# Autodesk Inventor assembly: 部件1
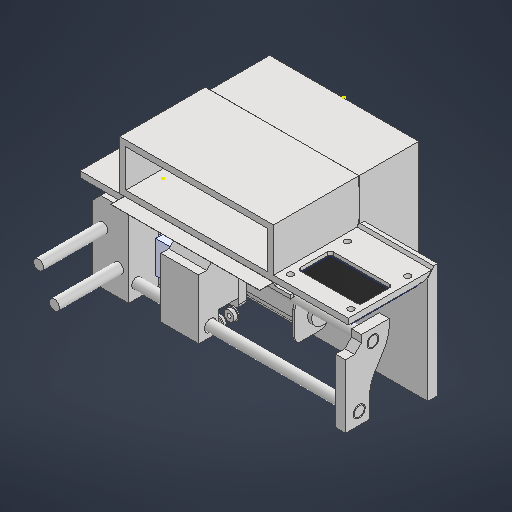
[picture p0: Inventor's stored thumbnail of the model, 512x512]
Saved by Autodesk Inventor 2025 (Build 290162000, 162)
## iProperties
Created: 2025-11-30
Part Number: 部件1
Document SubType Name: Assembly
Designer: XH
Author: XH
## Documents named in this file (11)
- C:\1A_Engineering_files\braille-printer-v2\部件1.iam
- C:\1A_Engineering_files\braille-printer-v2\便签.ipt
- C:\1A_Engineering_files\braille-printer-v2\主体.ipt
- C:\1A_Engineering_files\braille-printer-v2\前舵机位置控制.ipt
- C:\1A_Engineering_files\braille-printer-v2\针头主体.iam
- C:\1A_Engineering_files\braille-printer-v2\钢轴.ipt
- C:\1A_Engineering_files\braille-printer-v2\Y轴杠轴.ipt
- C:\1A_Engineering_files\braille-printer-v2\xy转接连杆.ipt
- C:\1A_Engineering_files\braille-printer-v2\阻挡X轴.ipt
- C:\1A_Engineering_files\braille-printer-v2\AZ-Delivery - OLED13 IIC.ipt
- C:\1A_Engineering_files\braille-printer-v2\大外壳.ipt
## Components (12 placed, 10 different names)
1. 便签:1 — 配合:1, 配合:2
2. 主体:1 — 配合:1, 配合:2, 表面齐平:7, 配合:12, 配合:13, 表面齐平:9, 配合:17, 表面齐平:10, 表面齐平:11
3. 前舵机位置控制:1 — 配合:14, 配合:15, 配合:16, 表面齐平:9
4. 针头主体:1 [sub-assembly] — 配合:4, 配合:5
5. 钢轴:1 — 表面齐平:3, 配合:4, 配合:6, 配合:10
6. 钢轴:2 — 表面齐平:3, 配合:5, 配合:7, 表面齐平:8, 配合:11
7. Y轴杠轴:1 — 表面齐平:5, 配合:8, 配合:13
8. Y轴杠轴:2 — 表面齐平:5, 配合:9, 配合:12
9. xy转接连杆:1 — 配合:6, 配合:7, 表面齐平:7, 配合:8, 配合:9
10. 阻挡X轴:1 — 表面齐平:8, 配合:10, 配合:11
11. AZ-Delivery - OLED13 IIC:1 — 配合:14, 配合:15, 配合:16
12. 大外壳:1 — 配合:17, 表面齐平:10, 表面齐平:11
## Relationships (23: Mate 16, Flush 7)
- 配合:1 [Mate]: 便签:1 ↔ 主体:1
- 配合:2 [Mate]: 便签:1 ↔ 主体:1
- 表面齐平:3 [Flush]: 钢轴:1 ↔ 钢轴:2
- 配合:4 [Mate]: 针头主体:1 ↔ 钢轴:1
- 配合:5 [Mate]: 针头主体:1 ↔ 钢轴:2
- 表面齐平:5 [Flush]: Y轴杠轴:1 ↔ Y轴杠轴:2
- 配合:6 [Mate]: 钢轴:1 ↔ xy转接连杆:1
- 配合:7 [Mate]: 钢轴:2 ↔ xy转接连杆:1
- 表面齐平:7 [Flush]: 主体:1 ↔ xy转接连杆:1
- 配合:8 [Mate]: Y轴杠轴:1 ↔ xy转接连杆:1
- 配合:9 [Mate]: Y轴杠轴:2 ↔ xy转接连杆:1
- 表面齐平:8 [Flush]: 钢轴:2 ↔ 阻挡X轴:1
- 配合:10 [Mate]: 钢轴:1 ↔ 阻挡X轴:1
- 配合:11 [Mate]: 钢轴:2 ↔ 阻挡X轴:1
- 配合:12 [Mate]: 主体:1 ↔ Y轴杠轴:2
- 配合:13 [Mate]: 主体:1 ↔ Y轴杠轴:1
- 配合:14 [Mate]: 前舵机位置控制:1 ↔ AZ-Delivery - OLED13 IIC:1
- 配合:15 [Mate]: 前舵机位置控制:1 ↔ AZ-Delivery - OLED13 IIC:1
- 配合:16 [Mate]: 前舵机位置控制:1 ↔ AZ-Delivery - OLED13 IIC:1
- 表面齐平:9 [Flush]: 主体:1 ↔ 前舵机位置控制:1
- 配合:17 [Mate]: 主体:1 ↔ 大外壳:1
- 表面齐平:10 [Flush]: 主体:1 ↔ 大外壳:1
- 表面齐平:11 [Flush]: 主体:1 ↔ 大外壳:1
